# Autodesk Inventor assembly: Joule Heating-bnk
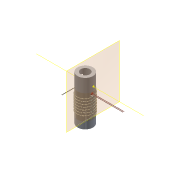
[picture p0: Inventor's stored thumbnail of the model, 180x180]
Saved by Autodesk Inventor 2017 (Build 210142000, 142)
## iProperties
Created: 2016-12-16
Part Number: Joule Heating-bnk
Description: STEP AP214
Document SubType Name: Assembly
Designer: br009491
Sending System: SolidWorks 2016
Preprocessor: SwSTEP 2.0
Title: Joule Heating.STEP
Revision Number: ANY
## Documents named in this file (5)
- C:\Users\ge937963\Desktop\Inventor View\Heating Block.iam
- C:\Users\ge937963\Desktop\Inventor View\Al Rod.ipt
- C:\Users\ge937963\Desktop\Inventor View\Tape.ipt
- C:\Users\ge937963\Desktop\Inventor View\Coil.ipt
- C:\Users\ge937963\Desktop\Inventor View\Thermistor.ipt
## Components (4 placed, 4 different names)
1. Al Rod Height A Cooling_1 — Mate:1, Mate:3, Mate:4, Mate:5, Mate:6, Tangent:1
2. Tape:1 — Mate:5
3. Coil:1 — Mate:1
4. Thermistor:1 — Mate:6, Tangent:1
## Relationships (6: Mate 5, Tangent 1)
- Mate:1: Al Rod Height A Cooling_1 ↔ Coil:1
- Mate:3: Al Rod Height A Cooling_1
- Mate:4: Al Rod Height A Cooling_1
- Mate:5 (-10.16 mm): Al Rod Height A Cooling_1 ↔ Tape:1
- Mate:6: Al Rod Height A Cooling_1 ↔ Thermistor:1
- Tangent:1: Al Rod Height A Cooling_1 ↔ Thermistor:1
